# Autodesk Inventor assembly: ASY MSC 002 отстойник осветлитель
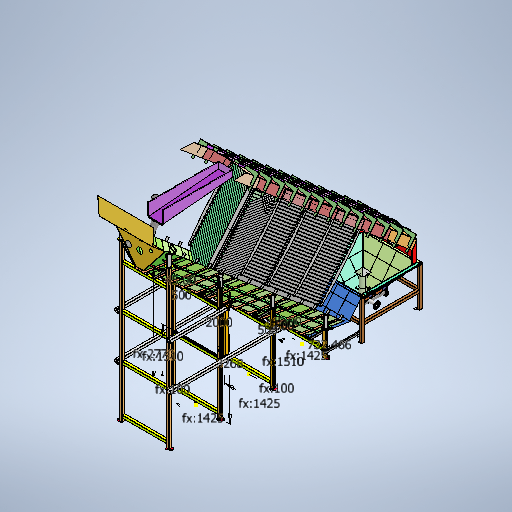
[picture p0: Inventor's stored thumbnail of the model, 512x512]
Saved by Autodesk Inventor 2025.1 (Build 291241020, 241B)
## iProperties
Created: 2024-09-05
Part Number: ASY MSC 002 отстойник осветлитель
Document SubType Name: Assembly
Designer: admin
Mass: 2.83156e+06 g
Surface Area: 4.02448e+06 cm^2
Volume: 367916 cm^3
Density: 7.69621 g/cm^3
Author: admin
## Documents named in this file (34)
- C:\Users\user\YandexDisk-badmisterfox\домашниий пк\Inventor\Manturovo\Manturovo_Se-clar\ASY MSC 002 отстойник осветлитель.iam
- C:\Users\user\YandexDisk-badmisterfox\домашниий пк\Inventor\Manturovo\Manturovo_Se-clar\ASY MSC 900.1 base frame.iam
- C:\Users\user\YandexDisk-badmisterfox\домашниий пк\Inventor\Manturovo\Manturovo_Se-clar\ASY MSC 100 cone.iam
- C:\Users\user\YandexDisk-badmisterfox\домашниий пк\Inventor\Manturovo\Manturovo_Se-clar\MSC 401 sheet lowerback.ipt
- C:\Users\user\YandexDisk-badmisterfox\домашниий пк\Inventor\Manturovo\Manturovo_Se-clar\MSC 701 face 1.ipt
- C:\Users\user\YandexDisk-badmisterfox\домашниий пк\Inventor\Manturovo\Manturovo_Se-clar\MSC 705 ridge 3.ipt
- C:\Users\user\YandexDisk-badmisterfox\домашниий пк\Inventor\Manturovo\Manturovo_Se-clar\MSC 713 tube.ipt
- C:\Users\user\YandexDisk-badmisterfox\домашниий пк\Inventor\Manturovo\Manturovo_Se-clar\ISO 5251 Bends 3D without straight ends(90 deg) DN150 11 11.ipt
- C:\Users\user\YandexDisk-badmisterfox\домашниий пк\Inventor\Manturovo\Manturovo_Se-clar\MSC 408 stringer lowerback.ipt
- C:\Users\user\YandexDisk-badmisterfox\домашниий пк\Inventor\Manturovo\Manturovo_Se-clar\MSC 703 face 2.ipt
- C:\Users\user\YandexDisk-badmisterfox\домашниий пк\Inventor\Manturovo\Manturovo_Se-clar\MSC 702 face 3.ipt
- C:\Users\user\YandexDisk-badmisterfox\домашниий пк\Inventor\Manturovo\Manturovo_Se-clar\MSC 704 face 4.ipt
- C:\Users\user\YandexDisk-badmisterfox\домашниий пк\Inventor\Manturovo\Manturovo_Se-clar\ASY MSC 900.3 base frame.iam
- C:\Users\user\YandexDisk-badmisterfox\домашниий пк\Inventor\Manturovo\Manturovo_Se-clar\Pillars\ASY MSC 900.5 base frame.iam
- C:\Users\user\YandexDisk-badmisterfox\домашниий пк\Inventor\Manturovo\Manturovo_Se-clar\Pillars\ASY MSC 900.4  base frame.iam
- C:\Users\user\YandexDisk-badmisterfox\домашниий пк\Inventor\Manturovo\Manturovo_Se-clar\Pillars\ASY MSC 900.6 base frame.iam
- C:\Users\user\YandexDisk-badmisterfox\домашниий пк\Inventor\Manturovo\Manturovo_Se-clar\ASY MSC 200 BACK.iam
- C:\Users\user\YandexDisk-badmisterfox\домашниий пк\Inventor\Manturovo\Manturovo_Se-clar\ASY MSC 300.2 LEFT BOARD.iam
- C:\Users\user\YandexDisk-badmisterfox\домашниий пк\Inventor\Manturovo\Manturovo_Se-clar\ASY MSC 300.1 RIGHT BOARD.iam
- C:\Users\user\YandexDisk-badmisterfox\домашниий пк\Inventor\Manturovo\Manturovo_Se-clar\ASY MSC 500 BELLY.iam
- C:\Users\user\YandexDisk-badmisterfox\домашниий пк\Inventor\Manturovo\Manturovo_Se-clar\ASY MSC 900.2 support.iam
- C:\Users\user\YandexDisk-badmisterfox\домашниий пк\Inventor\Manturovo\Manturovo_Se-clar\ASY MSC 600 cone exit back.iam
- C:\Users\user\YandexDisk-badmisterfox\домашниий пк\Inventor\Manturovo\Manturovo_Se-clar\ASY MSC 800 gills.iam
- C:\Users\user\YandexDisk-badmisterfox\домашниий пк\Inventor\Manturovo\Manturovo_Se-clar\ASY MSC 400 Accsess hatch.iam
- C:\Users\user\YandexDisk-badmisterfox\домашниий пк\Inventor\Manturovo\Manturovo_Se-clar\MSC DIM 000 settler-clarifier.ipt
- C:\Users\user\YandexDisk-badmisterfox\домашниий пк\Inventor\Manturovo\Manturovo_Se-clar\MSC DIM 001 frame.ipt
- C:\Users\user\YandexDisk-badmisterfox\домашниий пк\Inventor\Manturovo\Manturovo_Se-clar\ASY MSC 900.7 base frame transverse.iam
- C:\Users\user\YandexDisk-badmisterfox\домашниий пк\Inventor\Manturovo\Manturovo_Se-clar\ASY MSC 900.8 base frame transverse.iam
- C:\Users\user\YandexDisk-badmisterfox\домашниий пк\Inventor\Manturovo\Manturovo_Se-clar\MSC 908 transverse pillar plate.ipt
- C:\Users\user\YandexDisk-badmisterfox\домашниий пк\Inventor\Manturovo\Manturovo_Se-clar\MSC 900.9 base frame transverse.ipt
- C:\Users\user\YandexDisk-badmisterfox\домашниий пк\Inventor\Manturovo\Manturovo_Se-clar\ASY MSC 700 water tray.iam
- C:\Users\user\YandexDisk-badmisterfox\домашниий пк\Inventor\Manturovo\Manturovo_Se-clar\ASY 940 linkage.iam
- C:\Users\user\YandexDisk-badmisterfox\домашниий пк\Inventor\Manturovo\Manturovo_Se-clar\Part1.ipt
- C:\Users\user\YandexDisk-badmisterfox\домашниий пк\Inventor\Manturovo\Manturovo_Se-clar\ASY MSC 900.7 support.iam
## Components (52 placed, 35 different names)
1. MSC DIM 000 settler-clarifier.ipt:1
2. MSC DIM 001 frame.ipt:1
3. MSC 705 ridge 3.ipt:1
4. MSC 704 face 4.ipt:1
5. ASY MSC 300.2 LEFT BOARD.iam:1 [sub-assembly] — Rigid:11, Mate:34
6. ASY MSC 300.1 RIGHT BOARD.iam:1 [sub-assembly] — Rigid:10, Flush:17
7. MSC 908 transverse pillar plate.ipt:1
8. MSC 408 stringer lowerback.ipt:1
9. MSC 408 stringer lowerback.ipt:2
10. ASY MSC 400 Accsess hatch.iam:1 [sub-assembly] — Rigid:34
11. MSC 908 transverse pillar plate.ipt:2 — Mate:50, Flush:16, Flush:18
12. MSC 401 sheet lowerback.ipt:1 — Mate:29, Mate:30, Rigid:34
13. ASY MSC 100 cone.iam:1 [sub-assembly] — Mate:19, Flush:6, Mate:29, Rigid:17
14. ASY MSC 900.1 base frame.iam:1 [sub-assembly] — Flush:5, Mate:19, Mate:44, Mate:47, Mate:50, Flush:16
15. ASY 940 linkage.iam:2 [sub-assembly] — Rigid:31
16. ASY MSC 900.2 support.iam:8 [sub-assembly]
17. ASY 940 linkage.iam:1 [sub-assembly] — Rigid:32, Flush:18
18. Part1.ipt:1 — Rigid:33, Mate:68, Mate:69, Mate:70
19. MSC 900.9 base frame transverse.ipt:3 — Mate:68, Mate:69, Mate:70
20. ASY MSC 900.7 support:1 [sub-assembly] — Cylindrical:8, Mate:77
21. ASY MSC 900.3 base frame.iam:1 [sub-assembly] — Mate:23, Mate:24, Mate:44, Mate:45, Rigid:31, Rigid:32, Rigid:33, Cylindrical:8
22. ASY MSC 600 cone exit back.iam:1 [sub-assembly] — Rigid:17
23. Part1:2 — Mate:81, Mate:82
24. MSC 900.9 base frame transverse.ipt:4 — Mate:81, Mate:83
25. ASY MSC 900.7 support:2 [sub-assembly] — Cylindrical:11, Mate:78
26. ASY MSC 900.2 support.iam:5 [sub-assembly]
27. ASY MSC 900.4  base frame.iam:1 [sub-assembly] — Mate:32, Mate:33, Mate:45, Mate:46, Cylindrical:11, Mate:82
28. MSC 900.9 base frame transverse:7 — Mate:87, Mate:88
29. Part1:4 — Mate:88
30. ASY MSC 900.7 base frame transverse.iam:2 [sub-assembly] — Rigid:20
31. ASY MSC 900.7 base frame transverse.iam:1 [sub-assembly] — Rigid:19
32. ASY MSC 900.5 base frame.iam:1 [sub-assembly] — Flush:11, Cylindrical:7, Mate:46, Mate:48, Cylindrical:10
33. ASY MSC 200 BACK.iam:1 [sub-assembly] — Flush:8
34. ASY MSC 900.2 support.iam:4 [sub-assembly] — Cylindrical:7, Mate:41
35. ASY MSC 900.7 support:3 [sub-assembly] — Cylindrical:10, Mate:79
36. Part1:3 — Mate:84, Mate:85
37. MSC 900.9 base frame transverse.ipt:1 — Mate:85, Mate:86
38. MSC 900.9 base frame transverse.ipt:2
39. ASY MSC 900.7 support:4 [sub-assembly] — Cylindrical:9, Mate:80
40. MSC 713 tube.ipt:1 — Rigid:4
41. ISO 5251 Bends 3D without straight ends(90 deg) DN150 11 11.ipt:1
42. MSC 713 tube.ipt:2
43. MSC 703 face 2.ipt:1 — Flush:13, Flush:17, Mate:66
44. MSC 702 face 3.ipt:1 — Mate:34, Mate:35, Mate:36, Mate:66
45. ASY MSC 900.2 support.iam:1 [sub-assembly] — Cylindrical:6, Mate:42
46. MSC 701 face 1.ipt:1 — Rigid:4, Flush:9, Mate:35
47. ASY MSC 700 water tray.iam:1 [sub-assembly]
48. ASY MSC 500 BELLY.iam:1 [sub-assembly] — Flush:7, Mate:22, Rigid:10, Rigid:11, Mate:41, Mate:42, Mate:77, Mate:78, Mate:79, Mate:80, Mate:83, Mate:86, Mate:87
49. ASY MSC 900.6 base frame.iam:1 [sub-assembly] — Mate:38, Mate:39, Cylindrical:6, Mate:47, Rigid:19, Rigid:20, Rigid:21, Rigid:22, Cylindrical:9, Mate:84
50. ASY MSC 800 gills.iam:1 [sub-assembly] — Mate:22
51. ASY MSC 900.8 base frame transverse.iam:1 [sub-assembly] — Rigid:22
52. ASY MSC 900.8 base frame transverse.iam:2 [sub-assembly] — Rigid:21
## Relationships (85: Mate 47, WeldJoint 17, Flush 12, CylindricalJoint 8, RevoluteJoint 1)
- [Mate]: MSC 401 sheet lowerback.ipt:1 ↔ ASY MSC 100 cone.iam:1
- [WeldJoint]: MSC 713 tube.ipt:1 ↔ ISO 5251 Bends 3D without straight ends(90 deg) DN150 11 11.ipt:1
- [Mate]: MSC 408 stringer lowerback.ipt:1 ↔ ASY MSC 100 cone.iam:1
- [RevoluteJoint]: ISO 5251 Bends 3D without straight ends(90 deg) DN150 11 11.ipt:1 ↔ MSC 713 tube.ipt:2
- Rigid:4 [WeldJoint]: MSC 713 tube.ipt:1 ↔ MSC 701 face 1.ipt:1
- [Mate]: MSC 408 stringer lowerback.ipt:2 ↔ ASY MSC 100 cone.iam:1
- [Mate]: ASY MSC 600 cone exit back.iam:1 ↔ ASY MSC 500 BELLY.iam:1
- [WeldJoint]: MSC 705 ridge 3.ipt:1 ↔ ASY MSC 700 water tray.iam:1
- [WeldJoint]: MSC 705 ridge 3.ipt:1 ↔ ASY MSC 700 water tray.iam:1
- [Flush]: ASY MSC 600 cone exit back.iam:1 ↔ ASY MSC 500 BELLY.iam:1
- [Mate]: ASY MSC 500 BELLY.iam:1 ↔ ASY MSC 800 gills.iam:1
- [Mate]: MSC 701 face 1.ipt:1 ↔ ASY MSC 500 BELLY.iam:1
- [Mate] (-5 mm): MSC 701 face 1.ipt:1 ↔ ASY MSC 500 BELLY.iam:1
- [Mate] (3 mm): ASY MSC 900.2 support.iam:5 ↔ ASY MSC 500 BELLY.iam:1
- [Mate] (3 mm): ASY MSC 900.2 support.iam:8 ↔ ASY MSC 500 BELLY.iam:1
- [CylindricalJoint]: ASY MSC 900.2 support.iam:5 ↔ ASY MSC 900.4  base frame.iam:1
- [Mate] (-2860 mm): ASY MSC 200 BACK.iam:1 ↔ ASY MSC 500 BELLY.iam:1
- [CylindricalJoint]: ASY MSC 900.2 support.iam:8 ↔ ASY MSC 900.3 base frame.iam:1
- [Flush]: ASY MSC 900.3 base frame.iam:1 ↔ ASY MSC 900.4  base frame.iam:1
- Flush:5: ASY MSC 900.1 base frame.iam:1
- Mate:19: ASY MSC 100 cone.iam:1 ↔ ASY MSC 900.1 base frame.iam:1
- Flush:6: ASY MSC 100 cone.iam:1
- Flush:7: ASY MSC 500 BELLY.iam:1
- Flush:8: ASY MSC 200 BACK.iam:1
- Mate:22: ASY MSC 500 BELLY.iam:1 ↔ ASY MSC 800 gills.iam:1
- Mate:23: ASY MSC 900.3 base frame.iam:1
- Mate:24: ASY MSC 900.3 base frame.iam:1
- Flush:9: MSC 701 face 1.ipt:1
- Mate:29: MSC 401 sheet lowerback.ipt:1 ↔ ASY MSC 100 cone.iam:1
- Mate:30: MSC 401 sheet lowerback.ipt:1
- Rigid:10 [WeldJoint] (-25 mm): ASY MSC 300.1 RIGHT BOARD.iam:1 ↔ ASY MSC 500 BELLY.iam:1
- Rigid:11 [WeldJoint] (-25 mm): ASY MSC 300.2 LEFT BOARD.iam:1 ↔ ASY MSC 500 BELLY.iam:1
- Flush:11: ASY MSC 900.5 base frame.iam:1
- Mate:32: ASY MSC 900.4  base frame.iam:1
- Mate:33: ASY MSC 900.4  base frame.iam:1
- Mate:34: ASY MSC 300.2 LEFT BOARD.iam:1 ↔ MSC 702 face 3.ipt:1
- Mate:35: MSC 702 face 3.ipt:1 ↔ MSC 701 face 1.ipt:1
- [WeldJoint]: MSC 705 ridge 3.ipt:1 ↔ ASY MSC 700 water tray.iam:1
- Mate:36: MSC 702 face 3.ipt:1
- Mate:38: ASY MSC 900.6 base frame.iam:1
- Mate:39: ASY MSC 900.6 base frame.iam:1
- Cylindrical:6: ASY MSC 900.2 support.iam:1 ↔ ASY MSC 900.6 base frame.iam:1
- Cylindrical:7: ASY MSC 900.5 base frame.iam:1 ↔ ASY MSC 900.2 support.iam:4
- Mate:41 (3 mm): ASY MSC 900.2 support.iam:4 ↔ ASY MSC 500 BELLY.iam:1
- Mate:42 (3 mm): ASY MSC 900.2 support.iam:1 ↔ ASY MSC 500 BELLY.iam:1
- Flush:13: MSC 703 face 2.ipt:1
- Mate:44 (820 mm): ASY MSC 900.1 base frame.iam:1 ↔ ASY MSC 900.3 base frame.iam:1
- Mate:45 (1430 mm): ASY MSC 900.3 base frame.iam:1 ↔ ASY MSC 900.4  base frame.iam:1
- Mate:46 (1430 mm): ASY MSC 900.4  base frame.iam:1 ↔ ASY MSC 900.5 base frame.iam:1
- Mate:47 (5300 mm): ASY MSC 900.1 base frame.iam:1 ↔ ASY MSC 900.6 base frame.iam:1
- Rigid:17 [WeldJoint]: ASY MSC 100 cone.iam:1 ↔ ASY MSC 600 cone exit back.iam:1
- Mate:48: ASY MSC 900.5 base frame.iam:1
- Rigid:19 [WeldJoint]: ASY MSC 900.7 base frame transverse.iam:1 ↔ ASY MSC 900.6 base frame.iam:1
- Rigid:20 [WeldJoint]: ASY MSC 900.7 base frame transverse.iam:2 ↔ ASY MSC 900.6 base frame.iam:1
- Rigid:21 [WeldJoint]: ASY MSC 900.6 base frame.iam:1 ↔ ASY MSC 900.8 base frame transverse.iam:2
- Rigid:22 [WeldJoint]: ASY MSC 900.6 base frame.iam:1 ↔ ASY MSC 900.8 base frame transverse.iam:1
- Mate:50: MSC 908 transverse pillar plate.ipt:2 ↔ ASY MSC 900.1 base frame.iam:1
- Flush:16 (-40 mm): MSC 908 transverse pillar plate.ipt:2 ↔ ASY MSC 900.1 base frame.iam:1
- Flush:17: ASY MSC 300.1 RIGHT BOARD.iam:1 ↔ MSC 703 face 2.ipt:1
- Mate:66: MSC 703 face 2.ipt:1 ↔ MSC 702 face 3.ipt:1
- [WeldJoint]: MSC 908 transverse pillar plate.ipt:1 ↔ ASY 940 linkage.iam:2
- Rigid:31 [WeldJoint]: ASY 940 linkage.iam:2 ↔ ASY MSC 900.3 base frame.iam:1
- Rigid:32 [WeldJoint]: ASY 940 linkage.iam:1 ↔ ASY MSC 900.3 base frame.iam:1
- Flush:18: MSC 908 transverse pillar plate.ipt:2 ↔ ASY 940 linkage.iam:1
- Rigid:33 [WeldJoint]: Part1.ipt:1 ↔ ASY MSC 900.3 base frame.iam:1
- Mate:68: Part1.ipt:1 ↔ MSC 900.9 base frame transverse.ipt:3
- Mate:69 (11 mm): Part1.ipt:1 ↔ MSC 900.9 base frame transverse.ipt:3
- Mate:70: Part1.ipt:1 ↔ MSC 900.9 base frame transverse.ipt:3
- Cylindrical:8: ASY MSC 900.7 support:1 ↔ ASY MSC 900.3 base frame.iam:1
- Mate:77: ASY MSC 900.7 support:1 ↔ ASY MSC 500 BELLY.iam:1
- Cylindrical:9: ASY MSC 900.7 support:4 ↔ ASY MSC 900.6 base frame.iam:1
- Cylindrical:10: ASY MSC 900.5 base frame.iam:1 ↔ ASY MSC 900.7 support:3
- Cylindrical:11: ASY MSC 900.7 support:2 ↔ ASY MSC 900.4  base frame.iam:1
- Mate:78: ASY MSC 900.7 support:2 ↔ ASY MSC 500 BELLY.iam:1
- Mate:79: ASY MSC 900.7 support:3 ↔ ASY MSC 500 BELLY.iam:1
- Mate:80: ASY MSC 900.7 support:4 ↔ ASY MSC 500 BELLY.iam:1
- Mate:81: Part1:2 ↔ MSC 900.9 base frame transverse.ipt:4
- Mate:82: Part1:2 ↔ ASY MSC 900.4  base frame.iam:1
- Mate:83: MSC 900.9 base frame transverse.ipt:4 ↔ ASY MSC 500 BELLY.iam:1
- Mate:84: Part1:3 ↔ ASY MSC 900.6 base frame.iam:1
- Mate:85: Part1:3 ↔ MSC 900.9 base frame transverse.ipt:1
- Mate:86: MSC 900.9 base frame transverse.ipt:1 ↔ ASY MSC 500 BELLY.iam:1
- Mate:87: MSC 900.9 base frame transverse:7 ↔ ASY MSC 500 BELLY.iam:1
- Mate:88: MSC 900.9 base frame transverse:7 ↔ Part1:4
- Rigid:34 [WeldJoint]: ASY MSC 400 Accsess hatch.iam:1 ↔ MSC 401 sheet lowerback.ipt:1
## Named parameters: d334_d122 = 0 mm
